# Autodesk Inventor assembly: Z Idle Assembly
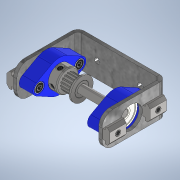
[picture p0: Inventor's stored thumbnail of the model, 180x180]
Saved by Autodesk Inventor 2022 (Build 260153000, 153)
## iProperties
Created: 2022-03-21
Part Number: Z Idle Assembly
Document SubType Name: Assembly
Designer: Nick
Author: Nick
## Documents named in this file (9)
- Y:\Projects\Bibble0\SubAsm\Z Idle Assembly.iam
- Y:\Projects\Bibble0\Sheet Metal\Z Idle Mount.ipt
- Y:\Projects\Bibble0\3D printed\Z Axis\Z Drive Bearing Holder.ipt
- Y:\Projects\Bibble0\Hardware\5 x 50mm Shaft.ipt
- Y:\Projects\Bibble0\Hardware\GT2 Pulley 16T.ipt
- Y:\Projects\Bibble0\Bearings\625 Bearing.ipt
- Y:\Projects\Bibble0\Hardware\M3 x 12 mm  SHCS.ipt
- Y:\Projects\Bibble0\Hardware\M3 T-Slot Nut.ipt
- Y:\Projects\Bibble0\Hardware\5mm Collar.ipt
## Components (16 placed, 8 different names)
1. Z Idle Mount:1 — Insert:12, Insert:13, Insert:14, Insert:15, Angle:2, Angle:4
2. Z Drive Bearing Holder:1 — Insert:8, Insert:9
3. Z Drive Bearing Holder:2 — Insert:10, Insert:11
4. 5 x 50mm Shaft:1 — Mate:2
5. GT2 Pulley 16T:1
6. 625 Bearing:1
7. 625 Bearing:2 — Mate:3
8. M3 x 12 mm  SHCS:1 — Insert:8
9. M3 x 12 mm  SHCS:2 — Insert:10
10. M3 x 12 mm  SHCS:3 — Insert:9
11. M3 x 12 mm  SHCS:4 — Insert:11
12. M3 T-Slot Nut:1 — Insert:12, Angle:3, Angle:4
13. M3 T-Slot Nut:2 — Insert:13, Angle:3
14. M3 T-Slot Nut:3 — Insert:14, Angle:1
15. M3 T-Slot Nut:4 — Insert:15, Angle:1, Angle:2
16. 5mm Collar:1 — Mate:2, Mate:3
## Relationships (23: Insert 15, Angle 4, Mate 3, Flush 1)
- [Mate]: 5 x 50mm Shaft:1 ↔ GT2 Pulley 16T:1
- [Insert]: Z Drive Bearing Holder:1 ↔ 625 Bearing:1
- [Insert]: Z Drive Bearing Holder:2 ↔ 625 Bearing:2
- [Insert]: GT2 Pulley 16T:1 ↔ 625 Bearing:1
- [Flush]: 5 x 50mm Shaft:1 ↔ 625 Bearing:2
- [Insert]: Z Idle Mount:1 ↔ Z Drive Bearing Holder:2
- [Insert]: Z Idle Mount:1 ↔ Z Drive Bearing Holder:2
- [Insert]: Z Idle Mount:1 ↔ Z Drive Bearing Holder:1
- [Insert]: Z Idle Mount:1 ↔ Z Drive Bearing Holder:1
- Insert:8: Z Drive Bearing Holder:1 ↔ M3 x 12 mm  SHCS:1
- Insert:9: Z Drive Bearing Holder:1 ↔ M3 x 12 mm  SHCS:3
- Insert:10: Z Drive Bearing Holder:2 ↔ M3 x 12 mm  SHCS:2
- Insert:11: Z Drive Bearing Holder:2 ↔ M3 x 12 mm  SHCS:4
- Insert:12: Z Idle Mount:1 ↔ M3 T-Slot Nut:1
- Insert:13: Z Idle Mount:1 ↔ M3 T-Slot Nut:2
- Insert:14: Z Idle Mount:1 ↔ M3 T-Slot Nut:3
- Insert:15: Z Idle Mount:1 ↔ M3 T-Slot Nut:4
- Angle:1 (0 deg): M3 T-Slot Nut:3 ↔ M3 T-Slot Nut:4
- Angle:2 (0 deg): Z Idle Mount:1 ↔ M3 T-Slot Nut:4
- Angle:3 (0 deg): M3 T-Slot Nut:1 ↔ M3 T-Slot Nut:2
- Angle:4 (0 deg): Z Idle Mount:1 ↔ M3 T-Slot Nut:1
- Mate:2: 5 x 50mm Shaft:1 ↔ 5mm Collar:1
- Mate:3: 625 Bearing:2 ↔ 5mm Collar:1
## Named parameters: d311_d223 = 0 mm
